# Autodesk Inventor assembly: ForeArm_hand
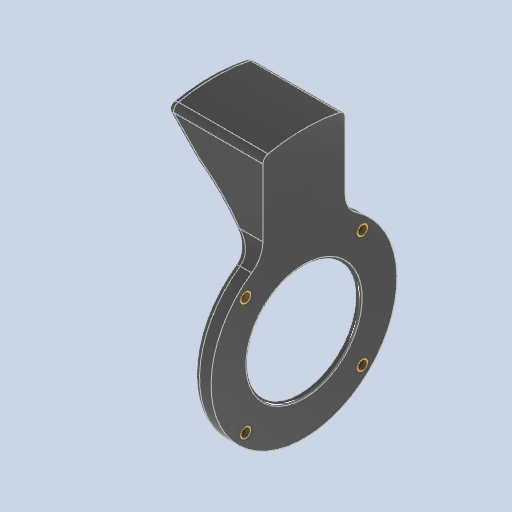
[picture p0: Inventor's stored thumbnail of the model, 512x512]
Saved by Autodesk Inventor 2022.3 (Build 263350000, 350)
## iProperties
Created: 2023-06-02
Part Number: ForeArm_hand
Document SubType Name: Assembly
Designer: Masato Kubotera
Author: Masato Kubotera
## Documents named in this file (3)
- C:\Users\Masato\Desktop\SUSTAINA-OP\UpperBody\Arm\ForeArm_hand.iam
- C:\Users\Masato\Desktop\SUSTAINA-OP\UpperBody\Arm\ForeArm_hand.ipt
- C:\Users\Masato\Desktop\SUSTAINA-OP\ReadyMade\InsertNut\UD-43040.ipt
## Components (5 placed, 2 different names)
1. UD-43040:1 — Insert:1
2. UD-43040:2 — Insert:2
3. UD-43040:3 — Insert:3
4. UD-43040:4 — Insert:4
5. ForeArm_hand:1 — Flush:1, Flush:2, Flush:3, Insert:1, Insert:2, Insert:3, Insert:4
## Relationships (7: Insert 4, Flush 3)
- Flush:1: ForeArm_hand:1
- Flush:2: ForeArm_hand:1
- Flush:3: ForeArm_hand:1
- Insert:1: UD-43040:1 ↔ ForeArm_hand:1
- Insert:2: UD-43040:2 ↔ ForeArm_hand:1
- Insert:3: UD-43040:3 ↔ ForeArm_hand:1
- Insert:4: UD-43040:4 ↔ ForeArm_hand:1
